# Autodesk Inventor assembly: Lead Screw Prototype A
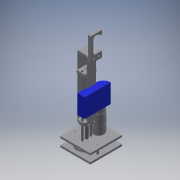
[picture p0: Inventor's stored thumbnail of the model, 180x180]
Saved by Autodesk Inventor 2019 (Build 230136000, 136)
## iProperties
Created: 2018-09-13
Part Number: Lead Screw Prototype A
Document SubType Name: Assembly
Designer: drawing
Author: drawing
## Documents named in this file (19)
- C:\Robotics\CAD\2018-19_CAD\lift\lift assembly\Lead Screw Prototype A.iam
- C:\Robotics\CAD\2018-19_CAD\lift\lift assembly\Part3.ipt
- C:\Robotics\CAD\2018-19_CAD\lift\lift assembly\ActoBotics Bearing .375.ipt
- C:\Robotics\CAD\2018-19_CAD\lift\lift assembly\Tetrix Gear 80T.ipt
- C:\Robotics\CAD\2018-19_CAD\lift\lift assembly\Part2.ipt
- C:\Robotics\CAD\2018-19_CAD\lift\lift assembly\Tetrix Gear 40T.ipt
- C:\Robotics\CAD\2018-19_CAD\lift\lift assembly\Part6.ipt
- C:\Robotics\CAD\2018-19_CAD\lift\lift assembly\Part5.ipt
- C:\Robotics\CAD\2018-19_CAD\lift\lift assembly\Andymark 2964  NeveRest 40 Motor.ipt
- C:\Robotics\CAD\2018-19_CAD\lift\lift assembly\AS 1420 - 1973 - M3 x 6.ipt
- C:\Robotics\CAD\2018-19_CAD\lift\lift assembly\ANSI B18.3 - 6-32 UNC - 0.5(31).ipt
- C:\Robotics\CAD\2018-19_CAD\lift\lift assembly\Tetrix Hub - axle.ipt
- C:\Robotics\CAD\2018-19_CAD\lift\lift assembly\Tetrix hub - motor.ipt
- C:\Robotics\CAD\2018-19_CAD\lift\lift assembly\Part11.ipt
- C:\Robotics\CAD\2018-19_CAD\lift\lift assembly\Part12.ipt
- C:\Robotics\CAD\2018-19_CAD\lift\lift assembly\lift top.ipt
- C:\Robotics\CAD\COTSParts\Fasteners\Nylon spacer .25.ipt
- C:\Robotics\CAD\2018-19_CAD\lift\hook.ipt
- C:\Robotics\CAD\2018-19_CAD\lift\lift holder.ipt
## Components (31 placed, 18 different names)
1. Part3:1 — Insert:1, Mate:3, Insert:10, Insert:11, Insert:13, Insert:14, Mate:8, Mate:9, Mate:10, Insert:15, Insert:16, Insert:17, Insert:18, Insert:19, Insert:20, Insert:21, Insert:22
2. ActoBotics Bearing .375:1 — Insert:1, Mate:11
3. Part3:2 — Insert:9, Insert:12, Mate:4
4. ActoBotics Bearing .375:2 — Insert:9
5. Tetrix Gear 80T:1 — Mate:1, Flush:1, Insert:26, Rotation/Translation:1, Rotation:1
6. Part2:1 — Mate:1, Mate:4, Mate:14, Mate:17, Flush:5
7. Tetrix Gear 40T:1 — Mate:3, Flush:1, Insert:27, Rotation:1
8. Part6:1 — Insert:10
9. Part6:2 — Insert:11, Insert:12
10. Part5:1 — Insert:13, Mate:15, Mate:18, Flush:4, Mate:22
11. Part5:2 — Insert:14, Mate:24
12. Andymark 2964  NeveRest 40 Motor:1 — Mate:8, Mate:9, Mate:10
13. AS 1420 - Metric M3 x 6:1 — Insert:19
14. AS 1420 - Metric M3 x 6:2 — Insert:17
15. AS 1420 - Metric M3 x 6:3 — Insert:18
16. AS 1420 - Metric M3 x 6:4 — Insert:20
17. AS 1420 - Metric M3 x 6:5 — Insert:15
18. AS 1420 - Metric M3 x 6:6 — Insert:16
19. Hexagon Socket Head Cap Screw - Inch No. 6 - 32 UNC - 1/2:1 — Insert:21
20. Hexagon Socket Head Cap Screw - Inch No. 6 - 32 UNC - 1/2:2 — Insert:22
21. Tetrix Hub - axle:1 — Insert:26, Mate:11
22. Tetrix hub - motor:1 — Insert:27
23. Part11:1 — Mate:16, Mate:19, Mate:20, Mate:23, Mate:26, Mate:27, Mate:28, Mate:29, Mate:32, Flush:6, Mate:33, Rotation/Translation:1
24. Hexagon Socket Head Cap Screw - Inch No. 6 - 32 UNC - 1/2:3 — Mate:21, Mate:22, Mate:23
25. Hexagon Socket Head Cap Screw - Inch No. 6 - 32 UNC - 1/2:4 — Mate:24, Mate:25
26. Part12:2 — Mate:14, Mate:15, Mate:16, Mate:19, Mate:20
27. lift top:1 — Mate:17, Mate:18, Flush:4, Flush:5, Mate:21, Mate:25
28. Nylon spacer .25:1 — Mate:28, Mate:29, Mate:31
29. Nylon spacer .25:2 — Mate:26, Mate:27, Mate:30, Mate:34
30. hook:1 — Mate:30, Mate:31, Mate:34
31. lift holder:1 — Mate:32, Flush:6, Mate:33
## Relationships (51: Mate 28, Insert 17, Flush 4, RelateRotateTranslate 1, RelateRotation 1)
- Insert:1: Part3:1 ↔ ActoBotics Bearing .375:1
- Mate:1: Tetrix Gear 80T:1 ↔ Part2:1
- Insert:9: Part3:2 ↔ ActoBotics Bearing .375:2
- Mate:3: Part3:1 ↔ Tetrix Gear 40T:1
- Flush:1: Tetrix Gear 80T:1 ↔ Tetrix Gear 40T:1
- Insert:10: Part3:1 ↔ Part6:1
- Insert:11: Part3:1 ↔ Part6:2
- Insert:12: Part3:2 ↔ Part6:2
- Mate:4: Part3:2 ↔ Part2:1
- Insert:13: Part3:1 ↔ Part5:1
- Insert:14: Part3:1 ↔ Part5:2
- Mate:8: Part3:1 ↔ Andymark 2964  NeveRest 40 Motor:1
- Mate:9: Part3:1 ↔ Andymark 2964  NeveRest 40 Motor:1
- Mate:10: Part3:1 ↔ Andymark 2964  NeveRest 40 Motor:1
- Insert:15: Part3:1 ↔ AS 1420 - Metric M3 x 6:5
- Insert:16: Part3:1 ↔ AS 1420 - Metric M3 x 6:6
- Insert:17: Part3:1 ↔ AS 1420 - Metric M3 x 6:2
- Insert:18: Part3:1 ↔ AS 1420 - Metric M3 x 6:3
- Insert:19: Part3:1 ↔ AS 1420 - Metric M3 x 6:1
- Insert:20: Part3:1 ↔ AS 1420 - Metric M3 x 6:4
- Insert:21: Part3:1 ↔ Hexagon Socket Head Cap Screw - Inch No. 6 - 32 UNC - 1/2:1
- Insert:22: Part3:1 ↔ Hexagon Socket Head Cap Screw - Inch No. 6 - 32 UNC - 1/2:2
- Insert:26: Tetrix Gear 80T:1 ↔ Tetrix Hub - axle:1
- Insert:27: Tetrix Gear 40T:1 ↔ Tetrix hub - motor:1
- Mate:11: ActoBotics Bearing .375:1 ↔ Tetrix Hub - axle:1
- Mate:14: Part2:1 ↔ Part12:2
- Mate:15: Part5:1 ↔ Part12:2
- Mate:16: Part11:1 ↔ Part12:2
- Mate:17: Part2:1 ↔ lift top:1
- Mate:18: Part5:1 ↔ lift top:1
- Flush:4: Part5:1 ↔ lift top:1
- Flush:5: Part2:1 ↔ lift top:1
- Mate:19: Part11:1 ↔ Part12:2
- Mate:20: Part11:1 ↔ Part12:2
- Mate:21: Hexagon Socket Head Cap Screw - Inch No. 6 - 32 UNC - 1/2:3 ↔ lift top:1
- Mate:22: Part5:1 ↔ Hexagon Socket Head Cap Screw - Inch No. 6 - 32 UNC - 1/2:3
- Mate:23: Part11:1 ↔ Hexagon Socket Head Cap Screw - Inch No. 6 - 32 UNC - 1/2:3
- Mate:24: Part5:2 ↔ Hexagon Socket Head Cap Screw - Inch No. 6 - 32 UNC - 1/2:4
- Mate:25: Hexagon Socket Head Cap Screw - Inch No. 6 - 32 UNC - 1/2:4 ↔ lift top:1
- Mate:26: Part11:1 ↔ Nylon spacer .25:2
- Mate:27: Part11:1 ↔ Nylon spacer .25:2
- Mate:28: Part11:1 ↔ Nylon spacer .25:1
- Mate:29: Part11:1 ↔ Nylon spacer .25:1
- Mate:30: Nylon spacer .25:2 ↔ hook:1
- Mate:31: Nylon spacer .25:1 ↔ hook:1
- Mate:32: Part11:1 ↔ lift holder:1
- Flush:6 (-50.8 mm): Part11:1 ↔ lift holder:1
- Mate:33: Part11:1 ↔ lift holder:1
- Mate:34: Nylon spacer .25:2 ↔ hook:1
- Rotation/Translation:1 [RelateRotateTranslate] (25.4 mm): Tetrix Gear 80T:1 ↔ Part11:1
- Rotation:1 [RelateRotation] (1 ul): Tetrix Gear 80T:1 ↔ Tetrix Gear 40T:1
